# Autodesk Inventor assembly: X95_XYZ_Stage_Large_Gate
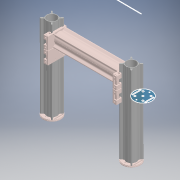
[picture p0: Inventor's stored thumbnail of the model, 180x180]
Saved by Autodesk Inventor 2019 (Build 230136000, 136)
## iProperties
Created: 2018-09-28
Part Number: X95_XYZ_Stage_Large_Gate
Document SubType Name: Assembly
Designer: voigt
Author: voigt
## Documents named in this file (4)
- D:\Microscope_Design\CAD_Files\mesoSPIM_design_V5.1\mesoSPIM\sample_stages\X95_XYZ_Stage_Large_Gate.iam
- D:\Microscope_Design\CAD_Files\mesoSPIM_design_V5.1\mesoSPIM\sample_stages\640mm_X95_with_base.iam
- D:\Microscope_Design\CAD_Files\mesoSPIM_design_V5.1\mesoSPIM\sample_stages\500mm_X95_crossmember_with_clamps.iam
- D:\Microscope_Design\CAD_Files\mesoSPIM_design_V5.1\library\Qioptiq\X95_carriers\X95_clamping_carrier.ipt
## Components (5 placed, 3 different names)
1. 640mm_X95_with_base:1 [sub-assembly] — Flush:1, Mate:1, Mate:9, Mate:10, Mate:11
2. 640mm_X95_with_base:2 [sub-assembly] — Flush:1, Mate:3, Flush:2, Mate:4, Mate:7, Mate:8
3. 500mm_X95_crossmember_with_clamps:1 [sub-assembly] — Mate:1, Mate:3, Flush:2, Mate:6, Mate:7, Mate:9, Mate:12
4. X95_clamping_carrier:1 — Mate:4, Mate:6, Mate:8
5. X95_clamping_carrier:2 — Mate:10, Mate:11, Mate:12
## Relationships (12: Mate 10, Flush 2)
- Flush:1: 640mm_X95_with_base:1 ↔ 640mm_X95_with_base:2
- Mate:1: 640mm_X95_with_base:1 ↔ 500mm_X95_crossmember_with_clamps:1
- Mate:3: 640mm_X95_with_base:2 ↔ 500mm_X95_crossmember_with_clamps:1
- Flush:2 (500 mm): 640mm_X95_with_base:2 ↔ 500mm_X95_crossmember_with_clamps:1
- Mate:4: 640mm_X95_with_base:2 ↔ X95_clamping_carrier:1
- Mate:6 (3 mm): 500mm_X95_crossmember_with_clamps:1 ↔ X95_clamping_carrier:1
- Mate:7: 640mm_X95_with_base:2 ↔ 500mm_X95_crossmember_with_clamps:1
- Mate:8: 640mm_X95_with_base:2 ↔ X95_clamping_carrier:1
- Mate:9: 640mm_X95_with_base:1 ↔ 500mm_X95_crossmember_with_clamps:1
- Mate:10: 640mm_X95_with_base:1 ↔ X95_clamping_carrier:2
- Mate:11: 640mm_X95_with_base:1 ↔ X95_clamping_carrier:2
- Mate:12 (3 mm): 500mm_X95_crossmember_with_clamps:1 ↔ X95_clamping_carrier:2
